# Autodesk Inventor assembly: Mockup_Omniscope_xiao
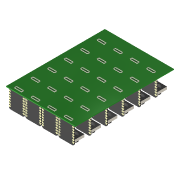
[picture p0: Inventor's stored thumbnail of the model, 180x180]
Saved by Autodesk Inventor 2022 (Build 260153000, 153)
## iProperties
Created: 2023-04-24
Part Number: Mockup_Omniscope_xiao
Document SubType Name: Assembly
Designer: diederichbenedict
Author: diederichbenedict
## Documents named in this file (3)
- C:\Users\diederichbenedict\Dropbox\Dokumente\Promotion\PROJECTS\Omniscope\INVENTOR\Mockup_Omniscope_xiao.iam
- C:\Users\diederichbenedict\Dropbox\Dokumente\Promotion\PROJECTS\Omniscope\INVENTOR\00_Seeeduino Xiao.ipt
- C:\Users\diederichbenedict\Dropbox\Dokumente\Promotion\PROJECTS\Omniscope\INVENTOR\00_PCB_Xiao_Camera_array.ipt
## Components (25 placed, 2 different names)
1. 00_PCB_Xiao_Camera_array:1 — Fluchtend:1
2. 00_Seeeduino Xiao:1
3. 00_Seeeduino Xiao:2
4. 00_Seeeduino Xiao:3
5. 00_Seeeduino Xiao:4
6. 00_Seeeduino Xiao:5
7. 00_Seeeduino Xiao:6
8. 00_Seeeduino Xiao:7
9. 00_Seeeduino Xiao:8
10. 00_Seeeduino Xiao:9
11. 00_Seeeduino Xiao:10
12. 00_Seeeduino Xiao:11
13. 00_Seeeduino Xiao:12
14. 00_Seeeduino Xiao:13
15. 00_Seeeduino Xiao:14
16. 00_Seeeduino Xiao:15
17. 00_Seeeduino Xiao:16
18. 00_Seeeduino Xiao:17
19. 00_Seeeduino Xiao:18
20. 00_Seeeduino Xiao:19
21. 00_Seeeduino Xiao:20
22. 00_Seeeduino Xiao:21
23. 00_Seeeduino Xiao:22
24. 00_Seeeduino Xiao:23
25. 00_Seeeduino Xiao:24 — Fluchtend:1
## Component patterns: (24 elements, first: 00_Seeeduino Xiao:1)
## Relationships (1: Flush 1)
- Fluchtend:1 [Flush]: 00_PCB_Xiao_Camera_array:1 ↔ 00_Seeeduino Xiao:24
